# Autodesk Inventor assembly: Schuss
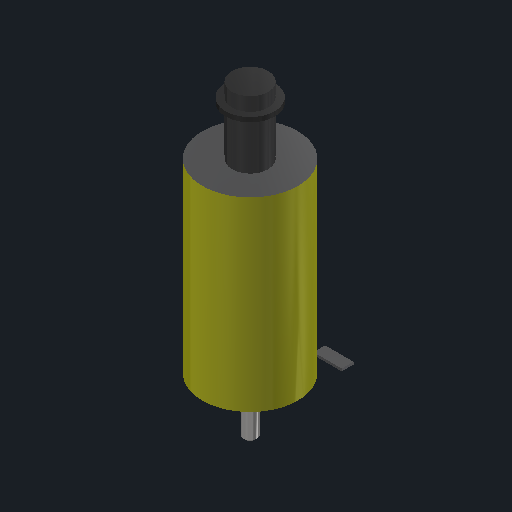
[picture p0: Inventor's stored thumbnail of the model, 512x512]
Saved by Autodesk Inventor 2023.2 (Build 272271030, 271C)
## iProperties
Created: 2018-01-28
Part Number: Schuss
Material: Generisch
Document SubType Name: Assembly
Designer: SoccerXY
Mass: 19.0948 g
Surface Area: 102.227 cm^2
Volume: 19.0948 cm^3
Density: 1 g/cm^3
Author: SoccerXY
## Documents named in this file (3)
- C:\Users\Elias Braun\Nextcloud2\RoboCup2023\Shoot\Schuss.iam
- C:\Users\Elias Braun\Nextcloud2\RoboCup2023\Shoot\Roboter2018Kolben.ipt
- C:\Users\Elias Braun\Nextcloud2\RoboCup2023\Shoot\Roboter2018Schuss.ipt
## Components (2 placed, 2 different names)
1. Roboter2018Kolben:1 — Passend:1
2. Roboter2018Schuss:1 — Passend:1
## Relationships (1: Mate 1)
- Passend:1 [Mate]: Roboter2018Kolben:1 ↔ Roboter2018Schuss:1
